# Autodesk Inventor assembly: Nozzle
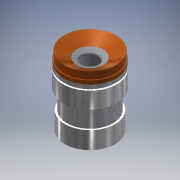
[picture p0: Inventor's stored thumbnail of the model, 180x180]
Saved by Autodesk Inventor 2017 (Build 210142000, 142)
## iProperties
Created: 2016-10-18
Part Number: Nozzle
Document SubType Name: Assembly
Designer: cflannery
Author: cflannery
## Documents named in this file (7)
- D:\Triton_Rocket_Club\Propulsion\Launches\8-inch-flight\Design\CAD\Nozzle\trunk\Nozzle.iam
- D:\Triton_Rocket_Club\Propulsion\Launches\8-inch-flight\Design\CAD\Nozzle\trunk\Aluminum_Carrier.ipt
- D:\Triton_Rocket_Club\Propulsion\Launches\8-inch-flight\Design\CAD\Nozzle\trunk\graphite.ipt
- D:\Triton_Rocket_Club\Propulsion\Launches\8-inch-flight\Design\CAD\Nozzle\trunk\Phenolic_cap.ipt
- D:\Triton_Rocket_Club\Propulsion\Launches\8-inch-flight\Design\CAD\Nozzle\trunk\Phenolic-liner.ipt
- D:\Triton_Rocket_Club\Propulsion\Launches\8-inch-flight\Design\CAD\Nozzle\trunk\retainer.ipt
- D:\Triton_Rocket_Club\Propulsion\Launches\8-inch-flight\Design\CAD\Nozzle\trunk\Skirt.ipt
## Components (6 placed, 6 different names)
1. Aluminum_Carrier:1 — Mate:5, Mate:6, Mate:7, Mate:8, Mate:9, Mate:10
2. graphite:1 — Mate:1, Mate:2, Mate:4
3. Phenolic_cap:1 — Mate:1, Mate:2, Mate:3, Mate:5, Mate:6
4. Phenolic-liner:1 — Mate:3, Mate:4
5. retainer:1 — Mate:7, Mate:9
6. Skirt:1 — Mate:8, Mate:10
## Relationships (10: Mate 10)
- Mate:1: graphite:1 ↔ Phenolic_cap:1
- Mate:2: graphite:1 ↔ Phenolic_cap:1
- Mate:3: Phenolic_cap:1 ↔ Phenolic-liner:1
- Mate:4: graphite:1 ↔ Phenolic-liner:1
- Mate:5: Aluminum_Carrier:1 ↔ Phenolic_cap:1
- Mate:6: Aluminum_Carrier:1 ↔ Phenolic_cap:1
- Mate:7: Aluminum_Carrier:1 ↔ retainer:1
- Mate:8: Aluminum_Carrier:1 ↔ Skirt:1
- Mate:9: Aluminum_Carrier:1 ↔ retainer:1
- Mate:10: Aluminum_Carrier:1 ↔ Skirt:1
